# Autodesk Inventor assembly: Motor Assembly
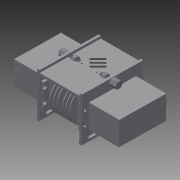
[picture p0: Inventor's stored thumbnail of the model, 180x180]
Saved by Autodesk Inventor 2014 SP1 (Build 180222100, 222)
## iProperties
Created: 2014-03-20
Part Number: Motor Assembly
Document SubType Name: Assembly
Designer: ehagerup
Author: ehagerup
## Documents named in this file (6)
- C:\Users\ehagerup\SkyDrive\Documents\Mechanical Sketches\Animatronic Tail V4\Motor Assembly.iam
- C:\Users\ehagerup\SkyDrive\Documents\Mechanical Sketches\Animatronic Tail V4\Whinch Servo.ipt
- C:\Users\ehagerup\SkyDrive\Documents\Mechanical Sketches\Animatronic Tail V4\Motor_Mount_Side.ipt
- C:\Users\ehagerup\SkyDrive\Documents\Mechanical Sketches\Animatronic Tail V4\Motor_Mount_Front.ipt
- C:\Users\ehagerup\Documents\Inventor\Content Center Files\R2014\en-US\ANSI B18.2.3.5M\ANSI B18.2.3.5M - M5 x 0.8 x 20.ipt
- C:\Users\ehagerup\Documents\Inventor\Content Center Files\R2014\en-US\ANSI B 18.2.4.1 M(1)\ANSI B 18.2.4.1 M - M5 x 0.8Style 1.ipt
## Components (11 placed, 5 different names)
1. Whinch Servo:1 — Flush:1, Flush:2, Mate:1, Mate:2, Mate:4
2. Whinch Servo:2 — Flush:1, Flush:2, Mate:1, Mate:3, Mate:5
3. Motor_Mount_Side:1 — Flush:3, Flush:4, Mate:2, Mate:4, Mate:10, Mate:11
4. Motor_Mount_Side:2 — Flush:3, Flush:4, Mate:3, Mate:5, Flush:5, Flush:6, Mate:6, Mate:19, Mate:21
5. Motor_Mount_Front:1 — Flush:5, Flush:6, Mate:6, Mate:12, Mate:22
6. Hex Bolt - Metric M5 x 0.8 x 20:3 — Mate:17, Mate:18, Mate:20, Mate:21
7. Hex Bolt - Metric M5 x 0.8 x 20:4 — Mate:7, Mate:8, Mate:9, Mate:11
8. Hex Nut Metric M5 x 0.8:3 — Mate:17, Mate:19, Mate:20
9. Hex Nut Metric M5 x 0.8:4 — Mate:7, Mate:12
10. Hex Nut Metric M5 x 0.8:7 — Mate:18, Mate:22
11. Hex Nut Metric M5 x 0.8:8 — Mate:8, Mate:9, Mate:10
## Relationships (24: Mate 18, Flush 6)
- Flush:1: Whinch Servo:1 ↔ Whinch Servo:2
- Flush:2: Whinch Servo:1 ↔ Whinch Servo:2
- Mate:1 (45 mm): Whinch Servo:1 ↔ Whinch Servo:2
- Flush:3: Motor_Mount_Side:1 ↔ Motor_Mount_Side:2
- Flush:4: Motor_Mount_Side:1 ↔ Motor_Mount_Side:2
- Mate:2: Whinch Servo:1 ↔ Motor_Mount_Side:1
- Mate:3: Whinch Servo:2 ↔ Motor_Mount_Side:2
- Mate:4: Whinch Servo:1 ↔ Motor_Mount_Side:1
- Mate:5: Whinch Servo:2 ↔ Motor_Mount_Side:2
- Flush:5: Motor_Mount_Side:2 ↔ Motor_Mount_Front:1
- Flush:6: Motor_Mount_Side:2 ↔ Motor_Mount_Front:1
- Mate:6: Motor_Mount_Side:2 ↔ Motor_Mount_Front:1
- Mate:7: Hex Bolt - Metric M5 x 0.8 x 20:4 ↔ Hex Nut Metric M5 x 0.8:4
- Mate:8: Hex Bolt - Metric M5 x 0.8 x 20:4 ↔ Hex Nut Metric M5 x 0.8:8
- Mate:9: Hex Bolt - Metric M5 x 0.8 x 20:4 ↔ Hex Nut Metric M5 x 0.8:8
- Mate:10: Motor_Mount_Side:1 ↔ Hex Nut Metric M5 x 0.8:8
- Mate:11: Motor_Mount_Side:1 ↔ Hex Bolt - Metric M5 x 0.8 x 20:4
- Mate:12: Motor_Mount_Front:1 ↔ Hex Nut Metric M5 x 0.8:4
- Mate:17: Hex Bolt - Metric M5 x 0.8 x 20:3 ↔ Hex Nut Metric M5 x 0.8:3
- Mate:18: Hex Bolt - Metric M5 x 0.8 x 20:3 ↔ Hex Nut Metric M5 x 0.8:7
- Mate:19: Motor_Mount_Side:2 ↔ Hex Nut Metric M5 x 0.8:3
- Mate:20: Hex Bolt - Metric M5 x 0.8 x 20:3 ↔ Hex Nut Metric M5 x 0.8:3
- Mate:21: Motor_Mount_Side:2 ↔ Hex Bolt - Metric M5 x 0.8 x 20:3
- Mate:22: Motor_Mount_Front:1 ↔ Hex Nut Metric M5 x 0.8:7
